# Autodesk Inventor assembly: module_5gth935_1z09136118_4x5eth935
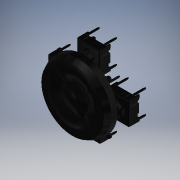
[picture p0: Inventor's stored thumbnail of the model, 180x180]
Saved by Autodesk Inventor 2017.3 (Build 213256000, 256)
## iProperties
Company: TraceParts S.A.
Created: 2018-03-09
Part Number: module_5gth935_1z09136118_4x5eth935
Checked By: TraceParts S.A.
Catalog Web Link: www.traceparts.com
Document SubType Name: Assembly
Designer: TraceParts
REFERENCE: 5GTH935+1Z09136118+4x5ETH935
DESIGN: 5G switch, through-hole mounting, 3,5N, black 1Z cap, pad printed, with legend on the edges, legend in the centre: OK, + 4 x 5E switches, through-hole mounting, 3,5N
SUPPLIER: MEC
TraceParts.PartNumber: 10-31052016-064422
TraceParts.PartTitle: Multimec Cap for a control unit - controlmec 5E/5G + 1Z
TraceParts.InstanceId: 10-31052016-064422ETEHLME269IU6PLDKLNAJUMSM
TraceParts.PartStatus: Published
TraceParts.PartVersion: 1.0.6
TRACEPARTS: TRACEPARTS
TraceParts.PartLanguage: en
TraceParts.ClassPath: MEC:/F_MEC/10-31052016-064422
Author: TraceParts
## Documents named in this file (6)
- C:\Users\Nils\Dropbox\THM\Eurobot\Display\IDF\70597241-9-module_5gth935_1z09136118_4x5eth935\module_5gth935_1z09136118_4x5eth935.iam
- C:\Users\Nils\Dropbox\THM\Eurobot\Display\IDF\70597241-9-module_5gth935_1z09136118_4x5eth935\module_5gth935_1z09136118_4x5eth935_01.ipt
- C:\Users\Nils\Dropbox\THM\Eurobot\Display\IDF\70597241-9-module_5gth935_1z09136118_4x5eth935\module_5gth935_1z09136118_4x5eth935_02.ipt
- C:\Users\Nils\Dropbox\THM\Eurobot\Display\IDF\70597241-9-module_5gth935_1z09136118_4x5eth935\module_5gth935_1z09136118_4x5eth935_03.ipt
- C:\Users\Nils\Dropbox\THM\Eurobot\Display\IDF\70597241-9-module_5gth935_1z09136118_4x5eth935\module_5gth935_1z09136118_4x5eth935_04.ipt
- C:\Users\Nils\Dropbox\THM\Eurobot\Display\IDF\70597241-9-module_5gth935_1z09136118_4x5eth935\module_5gth935_1z09136118_4x5eth935_05.ipt
## Components (5 placed, 5 different names)
1. module_5gth935_1z09136118_4x5eth935_02:1 — Fluchtend:1, Fluchtend:2
2. module_5gth935_1z09136118_4x5eth935_03:1
3. module_5gth935_1z09136118_4x5eth935_04:1
4. module_5gth935_1z09136118_4x5eth935_05:1
5. module_5gth935_1z09136118_4x5eth935_01:1
## Relationships (2: Flush 2)
- Fluchtend:1 [Flush] (-5 mm): module_5gth935_1z09136118_4x5eth935_02:1
- Fluchtend:2 [Flush] (-5 mm): module_5gth935_1z09136118_4x5eth935_02:1
